# Autodesk Inventor assembly: Condensers
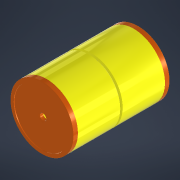
[picture p0: Inventor's stored thumbnail of the model, 180x180]
Saved by Autodesk Inventor 2022 (Build 260153000, 153)
## iProperties
Created: 2022-03-30
Part Number: Condensers
Document SubType Name: Assembly
Designer: Vinicius Miguel
Author: Vinicius Miguel
## Documents named in this file (4)
- C:\ViniFiles\SEM-Mechanical\Condensers.iam
- C:\ViniFiles\SEM-Mechanical\009.ipt
- C:\ViniFiles\SEM-Mechanical\010.ipt
- C:\ViniFiles\SEM-Mechanical\011.ipt
## Components (5 placed, 3 different names)
1. 009:1 — Mate:1, Flush:1, Mate:2, Mate:3
2. 009:2 — Mate:8, Mate:9
3. 010:1 — Mate:2, Mate:3, Mate:4, Mate:5, Mate:7
4. 010:2 — Mate:6, Mate:7, Mate:8, Mate:9
5. 011:1 — Mate:4, Mate:5, Mate:6
## Relationships (10: Mate 9, Flush 1)
- Mate:1: 009:1
- Flush:1: 009:1
- Mate:2: 009:1 ↔ 010:1
- Mate:3: 009:1 ↔ 010:1
- Mate:4: 010:1 ↔ 011:1
- Mate:5: 010:1 ↔ 011:1
- Mate:6: 010:2 ↔ 011:1
- Mate:7: 010:1 ↔ 010:2
- Mate:8: 009:2 ↔ 010:2
- Mate:9: 009:2 ↔ 010:2
